# Autodesk Inventor assembly: motor for rotation
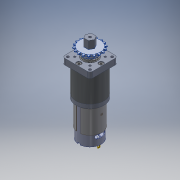
[picture p0: Inventor's stored thumbnail of the model, 180x180]
Saved by Autodesk Inventor 2018 (Build 220112000, 112)
## iProperties
Created: 2020-01-31
Part Number: motor for rotation
Document SubType Name: Assembly
Designer: s-2513225
Author: s-2513225
## Documents named in this file (3)
- \\studenthome\students\S-2513225\GitHub\2020CAD\Over bumper intake\Parts\motor for rotation.iam
- \\studenthome\students\S-2513225\GitHub\2020CAD\Over bumper intake\Parts\pg71 and 9015 motor and 1-2 hex output shaft.iam
- \\studenthome\students\S-2513225\GitHub\2020CAD\Over bumper intake\Parts\_18t_Aluminum_Hub_Sprocket_25_Chain_1_2_Hex_Bore_217-3488.ipt
## Components (2 placed, 2 different names)
1. pg71 and 9015 motor and 1-2 hex output shaft:1 [sub-assembly] — Flush:1, Mate:1
2. _18t_Aluminum_Hub_Sprocket_25_Chain_1_2_Hex_Bore_217-3488:1 — Flush:1, Mate:1
## Relationships (2: Flush 1, Mate 1)
- Flush:1 (12.7 mm): pg71 and 9015 motor and 1-2 hex output shaft:1 ↔ _18t_Aluminum_Hub_Sprocket_25_Chain_1_2_Hex_Bore_217-3488:1
- Mate:1: pg71 and 9015 motor and 1-2 hex output shaft:1 ↔ _18t_Aluminum_Hub_Sprocket_25_Chain_1_2_Hex_Bore_217-3488:1
